# Autodesk Inventor assembly: outer_mirrored
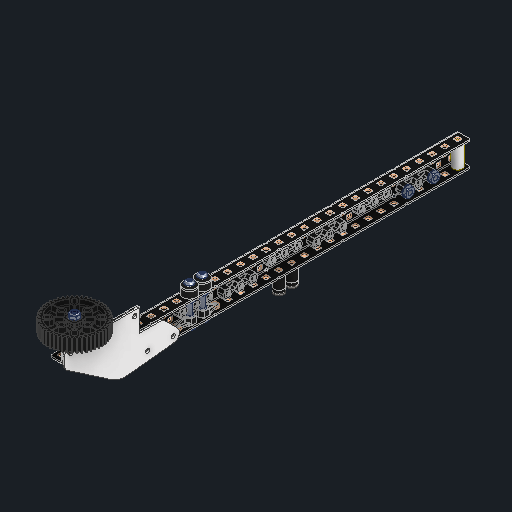
[picture p0: Inventor's stored thumbnail of the model, 512x512]
Saved by Autodesk Inventor 2024 (Build 280153000, 153)
## iProperties
Created: 2024-02-10
Part Number: outer_mirrored
Document SubType Name: Assembly
Designer: Averey Ku
Author: Averey Ku
## Documents named in this file (19)
- D:\vex_robotics\hardware\cad\vroomba_v0.1\chassis\drivebay\mirrored_parts\outer_mirrored.iam
- D:\vex_robotics\hardware\cad\vroomba_v0.1\chassis\drivebay\mirrored_parts\Alu C 1x2x1x28_mirrored.ipt
- D:\vex_robotics\hardware\cad\vroomba_v0.1\chassis\drivebay\mirrored_parts\Bearing Flat Low Profile_mirrored.ipt
- D:\vex_robotics\hardware\cad\vroomba_v0.1\chassis\drivebay\mirrored_parts\.375 OD Aluminum Spacer 0.875_mirrored.ipt
- D:\vex_robotics\hardware\cad\vroomba_v0.1\chassis\drivebay\mirrored_parts\Nut Keps_mirrored.ipt
- D:\vex_robotics\hardware\cad\vroomba_v0.1\chassis\drivebay\mirrored_parts\Nut Low Profile_mirrored.ipt
- D:\vex_robotics\hardware\cad\vroomba_v0.1\chassis\drivebay\mirrored_parts\1-Post Standoff Retainer_mirrored.ipt
- D:\vex_robotics\hardware\cad\VEX-CAD-Inventor-1.41\Motion\Spacers\Spacer Nylon .500 OD\NSpacer Black .500 OD x .250.ipt
- D:\vex_robotics\hardware\cad\VEX-CAD-Inventor-1.41\Motion\Spacers\Spacer Nylon .500 OD.ipt
- D:\vex_robotics\hardware\cad\vroomba_v0.1\chassis\drivebay\mirrored_parts\DWasher .500 OD x .062500_mirrored.ipt
- D:\vex_robotics\hardware\cad\VEX-CAD-Inventor-1.41\Structure\Hardware\Screw Shoulder Robosource\SScrew Shoulder Smooth 1.500 x .18.ipt
- D:\vex_robotics\hardware\cad\VEX-CAD-Inventor-1.41\Structure\Hardware\Screw Shoulder Robosource.ipt
- D:\vex_robotics\hardware\cad\vroomba_v0.1\chassis\drivebay\mirrored_parts\Nut Hex_mirrored.ipt
- D:\vex_robotics\hardware\cad\vroomba_v0.1\chassis\drivebay\mirrored_parts\rear_bumper_mirrored.iam
- D:\vex_robotics\hardware\cad\VEX-CAD-Inventor-1.41\Motion\Spacers\Spacer Nylon .375 OD\NSpacer .375 OD x .500.ipt
- D:\vex_robotics\hardware\cad\VEX-CAD-Inventor-1.41\Motion\Spacers\Spacer Nylon .375 OD.ipt
- D:\vex_robotics\hardware\cad\VEX-CAD-Inventor-1.41\Motion\Spacers\Spacer Nylon .375 OD\NSpacer .375 OD x .125.ipt
- D:\vex_robotics\hardware\cad\VEX-CAD-Inventor-1.41\Motion\Spacers\Washer Steel\SWasher .375 OD x .062500.ipt
- D:\vex_robotics\hardware\cad\VEX-CAD-Inventor-1.41\Motion\Spacers\Washer Steel.ipt
## Components (35 placed, 14 different names)
1. Alu C 1x2x1x28_mirrored:1 — Mate:1, Insert:1, Mate:2, Insert:2, Mate:3, Insert:3, Mate:4, Insert:4, Mate:5, Insert:5, Mate:6, Insert:6, Mate:7, Insert:7, Insert:8, Insert:9, Insert:14, Insert:15, Mate:9, Insert:21, Mate:8, Insert:20, Insert:25, Insert:24, Insert:28, Insert:29, Mate:10, Insert:34, Insert:33, Insert:34
2. Bearing Flat Low Profile_mirrored:1 — Mate:1, Insert:1, Insert:31, Insert:30
3. Bearing Flat Low Profile_mirrored:2 — Mate:2, Insert:2
4. Bearing Flat Low Profile_mirrored:3 — Mate:3, Insert:3
5. Bearing Flat Low Profile_mirrored:4 — Mate:4, Insert:4, Insert:33, Insert:32
6. Bearing Flat Low Profile_mirrored:5 — Mate:5, Insert:5
7. Bearing Flat Low Profile_mirrored:6 — Mate:6, Insert:6
8. Bearing Flat Low Profile_mirrored:7 — Mate:7, Insert:7
9. .375 OD Aluminum Spacer 0.875_mirrored:1 — Insert:8
10. .375 OD Aluminum Spacer 0.875_mirrored:2 — Insert:9
11. Nut Keps_mirrored:1 — Insert:14
12. Nut Keps_mirrored:2 — Insert:15
13. Nut Low Profile_mirrored:1 — Insert:19
14. Nut Low Profile_mirrored:2 — Insert:18
15. 1-Post Standoff Retainer_mirrored:1 — Mate:9, Insert:21, Insert:18
16. 1-Post Standoff Retainer_mirrored:2 — Mate:8, Insert:20, Insert:19
17. NSpacer Black .500 OD x .250:1 — Insert:25, Insert:23
18. NSpacer Black .500 OD x .250:2 — Insert:24, Insert:22
19. DWasher .500 OD x .062500_mirrored:1 — Insert:23, Insert:27
20. DWasher .500 OD x .062500_mirrored:2 — Insert:22, Insert:26
21. SScrew Shoulder Smooth 1.500 x .18:1 — Insert:27
22. SScrew Shoulder Smooth 1.500 x .18:2 — Insert:26
23. Nut Hex_mirrored:1 — Insert:28
24. Nut Hex_mirrored:2 — Insert:29
25. Nut Keps_mirrored:3 — Insert:31
26. Nut Keps_mirrored:4 — Insert:30
27. Nut Keps_mirrored:5 — Insert:33
28. Nut Keps_mirrored:6 — Insert:32
29. rear_bumper_mirrored:1 [sub-assembly] — Mate:10, Insert:34
30. NSpacer .375 OD x .500:1 — Insert:33
31. NSpacer .375 OD x .125:2
32. SWasher .375 OD x .062500:1
33. NSpacer .375 OD x .500:3 — Insert:34
34. NSpacer .375 OD x .125:4
35. SWasher .375 OD x .062500:2
## Relationships (44: Insert 34, Mate 10)
- Mate:1: Alu C 1x2x1x28_mirrored:1 ↔ Bearing Flat Low Profile_mirrored:1
- Insert:1: Alu C 1x2x1x28_mirrored:1 ↔ Bearing Flat Low Profile_mirrored:1
- Mate:2: Alu C 1x2x1x28_mirrored:1 ↔ Bearing Flat Low Profile_mirrored:2
- Insert:2: Alu C 1x2x1x28_mirrored:1 ↔ Bearing Flat Low Profile_mirrored:2
- Mate:3: Alu C 1x2x1x28_mirrored:1 ↔ Bearing Flat Low Profile_mirrored:3
- Insert:3: Alu C 1x2x1x28_mirrored:1 ↔ Bearing Flat Low Profile_mirrored:3
- Mate:4: Alu C 1x2x1x28_mirrored:1 ↔ Bearing Flat Low Profile_mirrored:4
- Insert:4: Alu C 1x2x1x28_mirrored:1 ↔ Bearing Flat Low Profile_mirrored:4
- Mate:5: Alu C 1x2x1x28_mirrored:1 ↔ Bearing Flat Low Profile_mirrored:5
- Insert:5: Alu C 1x2x1x28_mirrored:1 ↔ Bearing Flat Low Profile_mirrored:5
- Mate:6: Alu C 1x2x1x28_mirrored:1 ↔ Bearing Flat Low Profile_mirrored:6
- Insert:6: Alu C 1x2x1x28_mirrored:1 ↔ Bearing Flat Low Profile_mirrored:6
- Mate:7: Alu C 1x2x1x28_mirrored:1 ↔ Bearing Flat Low Profile_mirrored:7
- Insert:7: Alu C 1x2x1x28_mirrored:1 ↔ Bearing Flat Low Profile_mirrored:7
- Insert:8: Alu C 1x2x1x28_mirrored:1 ↔ .375 OD Aluminum Spacer 0.875_mirrored:1
- Insert:9: Alu C 1x2x1x28_mirrored:1 ↔ .375 OD Aluminum Spacer 0.875_mirrored:2
- Insert:14: Alu C 1x2x1x28_mirrored:1 ↔ Nut Keps_mirrored:1
- Insert:15: Alu C 1x2x1x28_mirrored:1 ↔ Nut Keps_mirrored:2
- Mate:9: Alu C 1x2x1x28_mirrored:1 ↔ 1-Post Standoff Retainer_mirrored:1
- Insert:21: Alu C 1x2x1x28_mirrored:1 ↔ 1-Post Standoff Retainer_mirrored:1
- Insert:18: Nut Low Profile_mirrored:2 ↔ 1-Post Standoff Retainer_mirrored:1
- Mate:8: Alu C 1x2x1x28_mirrored:1 ↔ 1-Post Standoff Retainer_mirrored:2
- Insert:20: Alu C 1x2x1x28_mirrored:1 ↔ 1-Post Standoff Retainer_mirrored:2
- Insert:19: Nut Low Profile_mirrored:1 ↔ 1-Post Standoff Retainer_mirrored:2
- Insert:25: Alu C 1x2x1x28_mirrored:1 ↔ NSpacer Black .500 OD x .250:1
- Insert:24: Alu C 1x2x1x28_mirrored:1 ↔ NSpacer Black .500 OD x .250:2
- Insert:23: NSpacer Black .500 OD x .250:1 ↔ DWasher .500 OD x .062500_mirrored:1
- Insert:22: NSpacer Black .500 OD x .250:2 ↔ DWasher .500 OD x .062500_mirrored:2
- Insert:27 (1.5875 mm): DWasher .500 OD x .062500_mirrored:1 ↔ SScrew Shoulder Smooth 1.500 x .18:1
- Insert:26 (1.5875 mm): DWasher .500 OD x .062500_mirrored:2 ↔ SScrew Shoulder Smooth 1.500 x .18:2
- Insert:28: Alu C 1x2x1x28_mirrored:1 ↔ Nut Hex_mirrored:1
- Insert:29: Alu C 1x2x1x28_mirrored:1 ↔ Nut Hex_mirrored:2
- Insert:31 (1.27 mm): Bearing Flat Low Profile_mirrored:1 ↔ Nut Keps_mirrored:3
- Insert:30 (1.27 mm): Bearing Flat Low Profile_mirrored:1 ↔ Nut Keps_mirrored:4
- Insert:33 (1.27 mm): Bearing Flat Low Profile_mirrored:4 ↔ Nut Keps_mirrored:5
- Insert:32 (1.27 mm): Bearing Flat Low Profile_mirrored:4 ↔ Nut Keps_mirrored:6
- Mate:10: Alu C 1x2x1x28_mirrored:1 ↔ rear_bumper_mirrored:1
- Insert:34: Alu C 1x2x1x28_mirrored:1 ↔ rear_bumper_mirrored:1
- [Insert]: NSpacer .375 OD x .125:2 ↔ SWasher .375 OD x .062500:1
- [Insert]: NSpacer .375 OD x .500:1 ↔ NSpacer .375 OD x .125:2
- [Insert]: NSpacer .375 OD x .125:4 ↔ SWasher .375 OD x .062500:2
- [Insert]: NSpacer .375 OD x .500:3 ↔ NSpacer .375 OD x .125:4
- Insert:33: Alu C 1x2x1x28_mirrored:1 ↔ NSpacer .375 OD x .500:1
- Insert:34: Alu C 1x2x1x28_mirrored:1 ↔ NSpacer .375 OD x .500:3
## Named parameters: d58_d55 = 0 mm, d59_d56 = 0 mm, d40_d58_d55 = 0 mm, d41_d59_d56 = 0 mm
